# Autodesk Inventor assembly: Ra-Manager_Montagem_Relays
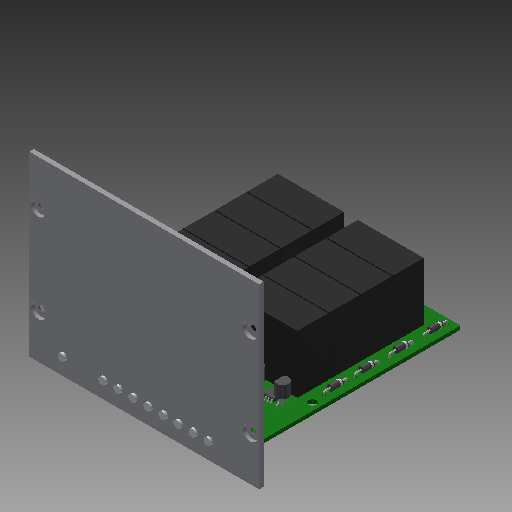
[picture p0: Inventor's stored thumbnail of the model, 512x512]
Saved by Autodesk Inventor 2019.4 (Build 234330000, 330)
## iProperties
Created: 2020-03-20
Part Number: Ra-Manager_Montagem_Relays
Material: Genérico
Document SubType Name: Assembly
Designer: caiom
Author: caiom
## Documents named in this file (4)
- C:\Users\caiom\Desktop\Ra-Manager_Mecanica\Ra-Manager_Montagem_Relays.iam
- C:\Users\caiom\Desktop\Ra-Manager_Mecanica\Ra-Manager_Painel-Placas_Relays.ipt
- C:\Users\caiom\Desktop\Ra-Manager_Mecanica\Ra-Manager_Light_Pipe.ipt
- C:\Users\caiom\Desktop\Ra-Manager_Mecanica\ExportSTEP\RA-Manager_Relays.ipt
## Components (11 placed, 3 different names)
1. Ra-Manager_Painel-Placas_Relays:1 — Coincidência:3, Coincidência:4, Coincidência:5, Coincidência:6, Coincidência:7, Coincidência:8, Coincidência:9, Coincidência:10, Coincidência:11, Alinhamento:1, Coincidência:12, Alinhamento:2
2. Ra-Manager_Light_Pipe:1 — Coincidência:3
3. Ra-Manager_Light_Pipe:2 — Coincidência:4
4. Ra-Manager_Light_Pipe:3 — Coincidência:5
5. Ra-Manager_Light_Pipe:4 — Coincidência:8
6. Ra-Manager_Light_Pipe:5 — Coincidência:9
7. Ra-Manager_Light_Pipe:6 — Coincidência:6
8. Ra-Manager_Light_Pipe:7 — Coincidência:7
9. Ra-Manager_Light_Pipe:8 — Coincidência:10
10. Ra-Manager_Light_Pipe:9 — Coincidência:11
11. RA-Manager_Relays:2 — Alinhamento:1, Coincidência:12, Alinhamento:2
## Relationships (13: Mate 11, Flush 2)
- Coincidência:2 [Mate]
- Coincidência:3 [Mate]: Ra-Manager_Painel-Placas_Relays:1 ↔ Ra-Manager_Light_Pipe:1
- Coincidência:4 [Mate]: Ra-Manager_Painel-Placas_Relays:1 ↔ Ra-Manager_Light_Pipe:2
- Coincidência:5 [Mate]: Ra-Manager_Painel-Placas_Relays:1 ↔ Ra-Manager_Light_Pipe:3
- Coincidência:6 [Mate]: Ra-Manager_Painel-Placas_Relays:1 ↔ Ra-Manager_Light_Pipe:6
- Coincidência:7 [Mate]: Ra-Manager_Painel-Placas_Relays:1 ↔ Ra-Manager_Light_Pipe:7
- Coincidência:8 [Mate]: Ra-Manager_Painel-Placas_Relays:1 ↔ Ra-Manager_Light_Pipe:4
- Coincidência:9 [Mate]: Ra-Manager_Painel-Placas_Relays:1 ↔ Ra-Manager_Light_Pipe:5
- Coincidência:10 [Mate]: Ra-Manager_Painel-Placas_Relays:1 ↔ Ra-Manager_Light_Pipe:8
- Coincidência:11 [Mate]: Ra-Manager_Painel-Placas_Relays:1 ↔ Ra-Manager_Light_Pipe:9
- Alinhamento:1 [Flush] (5.75 mm): Ra-Manager_Painel-Placas_Relays:1 ↔ RA-Manager_Relays:2
- Coincidência:12 [Mate] (2.75 mm): Ra-Manager_Painel-Placas_Relays:1 ↔ RA-Manager_Relays:2
- Alinhamento:2 [Flush] (10.7625 mm): Ra-Manager_Painel-Placas_Relays:1 ↔ RA-Manager_Relays:2
